# Autodesk Inventor assembly: dog_2
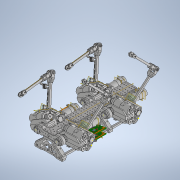
[picture p0: Inventor's stored thumbnail of the model, 180x180]
Saved by Autodesk Inventor 2020 (Build 240168000, 168)
## iProperties
Created: 2019-05-16
Part Number: dog_2
Document SubType Name: Assembly
Designer: psrob
Author: psrob
## Documents named in this file (18)
- E:\projects-2\project dog gen2\hardware\dog_2.iam
- E:\projects-2\project dog gen2\hardware\leg_ass_1.iam
- E:\projects-2\project dog gen2\hardware\carbon_fiber_200.ipt
- E:\projects-2\project dog gen2\hardware\leg_ass_1_MIR.iam
- E:\projects-2\project dog gen2\hardware\body_bone_1.ipt
- E:\projects-2\project dog gen2\hardware\body_bone_2.ipt
- E:\projects-2\project dog gen2\hardware\body_bone_3.ipt
- E:\projects-2\project dog gen2\hardware\body_bone_4.ipt
- E:\projects-2\project dog gen2\hardware\body_bone_5.ipt
- E:\projects-2\project dog gen2\hardware\body_carbon_fiber_holder_1.ipt
- E:\projects-2\project dog gen2\hardware\pcb_holder_1.ipt
- E:\projects-2\project dog gen2\hardware\pcb_holder_2.ipt
- E:\projects-2\project dog gen2\hardware\motor_holder_1.ipt
- E:\projects-2\project dog gen2\hardware\switch_holder_5.ipt
- E:\projects-2\project dog gen2\hardware\ele_3d_3\dog_driver_5.brd.iam
- E:\projects-2\project dog gen2\hardware\pcb_shell_n1.ipt
- E:\projects-2\project dog gen2\hardware\pcb_shell_n1_MIR.ipt
- E:\projects-2\project dog gen2\hardware\carbon_fiber_fixer_1.ipt
## Components (32 placed, 17 different names)
1. leg_ass_1:1 [sub-assembly] — Flush:2, Flush:3, Flush:4, Mate:4, Flush:8, Flush:9, Insert:6, Flush:14, Insert:8
2. leg_ass_1:2 [sub-assembly] — Flush:2, Flush:3, Flush:4, Mate:1, Mate:2, Flush:5, Mate:3, Flush:6, Flush:7, Flush:10, Flush:12, Insert:1, Insert:4, Insert:10, Insert:11, Flush:27
3. carbon_fiber_200:1 — Mate:1, Mate:2, Flush:5
4. leg_ass_1_MIR:1 [sub-assembly] — Mate:3, Flush:6, Flush:7, Insert:2, Insert:3, Flush:13, Insert:9, Insert:12, Tangent:1
5. leg_ass_1_MIR:2 [sub-assembly] — Mate:4, Flush:8, Flush:9, Flush:11, Insert:5, Insert:7
6. body_bone_1:1 — Flush:10, Insert:3, Insert:4, Insert:17, Insert:18, Insert:23, Insert:24
7. body_bone_2:1 — Flush:11, Insert:5, Insert:6, Insert:19, Insert:20, Insert:21, Insert:22
8. body_bone_3:1 — Flush:12, Insert:1, Insert:2
9. body_bone_4:1 — Flush:13, Insert:9, Insert:10, Insert:13, Insert:14, Insert:35, Insert:36
10. body_bone_5:1 — Flush:14, Insert:7, Insert:8, Mate:11, Flush:36, Insert:33, Insert:34
11. body_bone_1:2 — Insert:11, Insert:12, Insert:15, Insert:16, Flush:28, Insert:30, Angle:1, Insert:37
12. body_carbon_fiber_holder_1:1 — Flush:27, Insert:13, Insert:14, Mate:12, Flush:29, Mate:13, Flush:30, Mate:14, Mate:15, Flush:40
13. body_carbon_fiber_holder_1:2 — Insert:15, Insert:16
14. pcb_holder_1:1 — Flush:28, Insert:30, Flush:37, Insert:37, Mate:16, Flush:38, Insert:38, Insert:39, Insert:40, Insert:45, Insert:46, Insert:47, Insert:48
15. pcb_holder_2:1 — Mate:11
16. carbon_fiber_200:3 — Mate:13, Flush:30, Mate:14
17. carbon_fiber_200:4 — Mate:12, Flush:29, Mate:15
18. motor_holder_1:1 — Insert:17, Insert:18
19. motor_holder_1:2 — Insert:19, Insert:20
20. motor_holder_1:3 — Insert:23, Insert:24
21. motor_holder_1:4 — Insert:21, Insert:22
22. switch_holder_5:1 — Flush:36, Insert:33, Insert:34
23. switch_holder_5:2 — Insert:35, Insert:36
24. dog_driver_5.brd:1 [sub-assembly] — Flush:37, Angle:1, Tangent:1, Mate:16, Flush:39
25. pcb_shell_n1:1 — Flush:38, Flush:39, Insert:38
26. pcb_shell_n1_MIR:1 — Insert:39, Insert:40, Insert:41, Insert:42
27. dog_driver_5.brd:2 [sub-assembly] — Insert:41, Insert:42
28. pcb_shell_n1_MIR:2 — Insert:45, Insert:46
29. dog_driver_5.brd:3 [sub-assembly]
30. pcb_shell_n1:2 — Insert:47, Insert:48, Insert:49, Insert:50
31. dog_driver_5.brd:4 [sub-assembly] — Insert:49, Insert:50
32. carbon_fiber_fixer_1:1 — Flush:40
## Relationships (77: Insert 43, Flush 22, Mate 10, Angle 1, Tangent 1)
- Flush:2: leg_ass_1:1 ↔ leg_ass_1:2
- Flush:3 (180 mm): leg_ass_1:1 ↔ leg_ass_1:2
- Flush:4: leg_ass_1:1 ↔ leg_ass_1:2
- Mate:1: leg_ass_1:2 ↔ carbon_fiber_200:1
- Mate:2: leg_ass_1:2 ↔ carbon_fiber_200:1
- Flush:5 (10 mm): leg_ass_1:2 ↔ carbon_fiber_200:1
- Mate:3: leg_ass_1:2 ↔ leg_ass_1_MIR:1
- Flush:6: leg_ass_1:2 ↔ leg_ass_1_MIR:1
- Flush:7: leg_ass_1:2 ↔ leg_ass_1_MIR:1
- Mate:4: leg_ass_1:1 ↔ leg_ass_1_MIR:2
- Flush:8: leg_ass_1:1 ↔ leg_ass_1_MIR:2
- Flush:9: leg_ass_1:1 ↔ leg_ass_1_MIR:2
- Flush:10: leg_ass_1:2 ↔ body_bone_1:1
- Flush:11: leg_ass_1_MIR:2 ↔ body_bone_2:1
- Flush:12: leg_ass_1:2 ↔ body_bone_3:1
- Insert:1: leg_ass_1:2 ↔ body_bone_3:1
- Insert:2: leg_ass_1_MIR:1 ↔ body_bone_3:1
- Insert:3: leg_ass_1_MIR:1 ↔ body_bone_1:1
- Insert:4: leg_ass_1:2 ↔ body_bone_1:1
- Insert:5: leg_ass_1_MIR:2 ↔ body_bone_2:1
- Insert:6: leg_ass_1:1 ↔ body_bone_2:1
- Flush:13: leg_ass_1_MIR:1 ↔ body_bone_4:1
- Flush:14: leg_ass_1:1 ↔ body_bone_5:1
- Insert:7: leg_ass_1_MIR:2 ↔ body_bone_5:1
- Insert:8: leg_ass_1:1 ↔ body_bone_5:1
- Insert:9: leg_ass_1_MIR:1 ↔ body_bone_4:1
- Insert:10: leg_ass_1:2 ↔ body_bone_4:1
- Insert:11: leg_ass_1:2 ↔ body_bone_1:2
- Insert:12: leg_ass_1_MIR:1 ↔ body_bone_1:2
- Flush:27: leg_ass_1:2 ↔ body_carbon_fiber_holder_1:1
- Insert:13: body_bone_4:1 ↔ body_carbon_fiber_holder_1:1
- Insert:14: body_bone_4:1 ↔ body_carbon_fiber_holder_1:1
- Insert:15: body_bone_1:2 ↔ body_carbon_fiber_holder_1:2
- Insert:16: body_bone_1:2 ↔ body_carbon_fiber_holder_1:2
- Flush:28: body_bone_1:2 ↔ pcb_holder_1:1
- Mate:11: body_bone_5:1 ↔ pcb_holder_2:1
- Mate:12: body_carbon_fiber_holder_1:1 ↔ carbon_fiber_200:4
- Flush:29: body_carbon_fiber_holder_1:1 ↔ carbon_fiber_200:4
- Mate:13: body_carbon_fiber_holder_1:1 ↔ carbon_fiber_200:3
- Flush:30: body_carbon_fiber_holder_1:1 ↔ carbon_fiber_200:3
- Mate:14: body_carbon_fiber_holder_1:1 ↔ carbon_fiber_200:3
- Mate:15: body_carbon_fiber_holder_1:1 ↔ carbon_fiber_200:4
- Insert:17: body_bone_1:1 ↔ motor_holder_1:1
- Insert:18: body_bone_1:1 ↔ motor_holder_1:1
- Insert:19: body_bone_2:1 ↔ motor_holder_1:2
- Insert:20: body_bone_2:1 ↔ motor_holder_1:2
- Insert:21: body_bone_2:1 ↔ motor_holder_1:4
- Insert:22: body_bone_2:1 ↔ motor_holder_1:4
- Insert:23: body_bone_1:1 ↔ motor_holder_1:3
- Insert:24: body_bone_1:1 ↔ motor_holder_1:3
- Insert:30: body_bone_1:2 ↔ pcb_holder_1:1
- Flush:36: body_bone_5:1 ↔ switch_holder_5:1
- Insert:33: body_bone_5:1 ↔ switch_holder_5:1
- Insert:34: body_bone_5:1 ↔ switch_holder_5:1
- Insert:35: body_bone_4:1 ↔ switch_holder_5:2
- Insert:36: body_bone_4:1 ↔ switch_holder_5:2
- Flush:37 (-5 mm): pcb_holder_1:1 ↔ dog_driver_5.brd:1
- Angle:1 (170 deg): body_bone_1:2 ↔ dog_driver_5.brd:1
- Insert:37: body_bone_1:2 ↔ pcb_holder_1:1
- Tangent:1 (5 mm): leg_ass_1_MIR:1 ↔ dog_driver_5.brd:1
- Mate:16 (3 mm): pcb_holder_1:1 ↔ dog_driver_5.brd:1
- Flush:38: pcb_holder_1:1 ↔ pcb_shell_n1:1
- Flush:39: dog_driver_5.brd:1 ↔ pcb_shell_n1:1
- Insert:38: pcb_holder_1:1 ↔ pcb_shell_n1:1
- Insert:39: pcb_holder_1:1 ↔ pcb_shell_n1_MIR:1
- Insert:40: pcb_holder_1:1 ↔ pcb_shell_n1_MIR:1
- Insert:41: pcb_shell_n1_MIR:1 ↔ dog_driver_5.brd:2
- Insert:42: pcb_shell_n1_MIR:1 ↔ dog_driver_5.brd:2
- [Insert]: pcb_shell_n1_MIR:2 ↔ dog_driver_5.brd:3
- [Insert]: pcb_shell_n1_MIR:2 ↔ dog_driver_5.brd:3
- Insert:45: pcb_holder_1:1 ↔ pcb_shell_n1_MIR:2
- Insert:46: pcb_holder_1:1 ↔ pcb_shell_n1_MIR:2
- Insert:47: pcb_holder_1:1 ↔ pcb_shell_n1:2
- Insert:48: pcb_holder_1:1 ↔ pcb_shell_n1:2
- Insert:49: pcb_shell_n1:2 ↔ dog_driver_5.brd:4
- Insert:50: pcb_shell_n1:2 ↔ dog_driver_5.brd:4
- Flush:40: body_carbon_fiber_holder_1:1 ↔ carbon_fiber_fixer_1:1
## Named parameters: d142_d140 = 0 mm, d143_d141 = 0 mm
